# Autodesk Inventor assembly: Neck
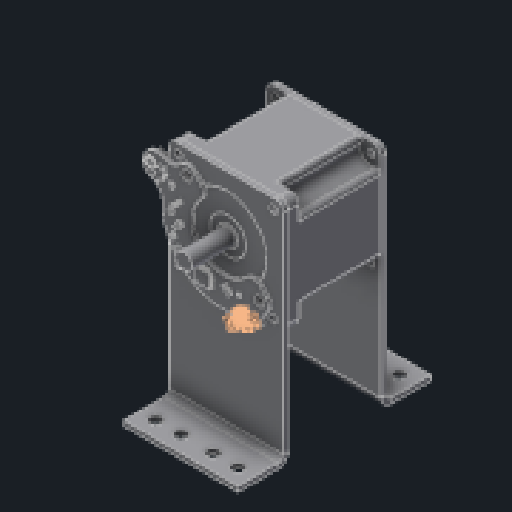
[picture p0: Inventor's stored thumbnail of the model, 512x512]
Saved by Autodesk Inventor 2025.2 (Build 292293000, 293)
## iProperties
Created: 2025-09-26
Part Number: Neck
Document SubType Name: Assembly
Designer: valer
Author: valer
## Documents named in this file (4)
- C:\Users\valer\Desktop\str1ker\cad\Neck.iam
- C:\Users\valer\Desktop\str1ker\cad\external\NeckMotor\SouluckNema23-0.7N-24V.ipt
- C:\Users\valer\Desktop\str1ker\cad\external\am-4179 Lamprey Absolute Encoder.ipt
- C:\Users\valer\Desktop\str1ker\cad\NeckStepperCover.ipt
## Components (4 placed, 3 different names)
1. SouluckNema23-0.7N-24V:1 — Mate:5, Mate:6, Mate:7, Mate:8, Mate:9, Mate:10
2. am-4179 Lamprey Absolute Encoder:1
3. NeckStepperCover:1
4. NeckStepperCover:2 — Mate:8, Mate:9, Mate:10
## Relationships (12: Mate 10, Flush 2)
- [Mate]: SouluckNema23-0.7N-24V:1 ↔ am-4179 Lamprey Absolute Encoder:1
- [Mate]: SouluckNema23-0.7N-24V:1 ↔ NeckStepperCover:1
- [Mate]: SouluckNema23-0.7N-24V:1 ↔ NeckStepperCover:1
- [Flush]: SouluckNema23-0.7N-24V:1 ↔ NeckStepperCover:1
- [Flush]: SouluckNema23-0.7N-24V:1 ↔ am-4179 Lamprey Absolute Encoder:1
- [Mate]: am-4179 Lamprey Absolute Encoder:1 ↔ NeckStepperCover:1
- Mate:5: SouluckNema23-0.7N-24V:1
- Mate:6: SouluckNema23-0.7N-24V:1
- Mate:7: SouluckNema23-0.7N-24V:1
- Mate:8: SouluckNema23-0.7N-24V:1 ↔ NeckStepperCover:2
- Mate:9: SouluckNema23-0.7N-24V:1 ↔ NeckStepperCover:2
- Mate:10: SouluckNema23-0.7N-24V:1 ↔ NeckStepperCover:2
